# Autodesk Inventor assembly: Pendolo_Inverso
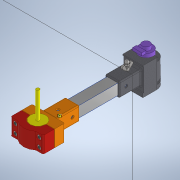
[picture p0: Inventor's stored thumbnail of the model, 180x180]
Saved by Autodesk Inventor 2020.2 (Build 242310000, 310)
## iProperties
Created: 2019-11-10
Part Number: Pendolo_Inverso
Document SubType Name: Assembly
Designer: socci
Mass: 329.019 g
Surface Area: 919.573 cm^2
Volume: 203.34 cm^3
Density: 1.61807 g/cm^3
Author: socci
## Documents named in this file (13)
- C:\Users\socci\Desktop\mv-Project\04_PartDraw\Assieme_Barra.iam
- C:\Users\socci\Desktop\mv-Project\04_PartDraw\Componenti\1_Asse_cuscinetti.ipt
- C:\Users\socci\Desktop\mv-Project\04_PartDraw\Componenti\2_Connettore_inf_sup.ipt
- C:\Users\socci\Desktop\mv-Project\04_PartDraw\Componenti\3_Connettore_inf_INF.ipt
- C:\Users\socci\Desktop\mv-Project\04_PartDraw\Componenti\4_barra.ipt
- C:\Users\socci\Desktop\mv-Project\04_PartDraw\Componenti\8_Connettore_sup.ipt
- C:\Users\socci\Desktop\mv-Project\04_PartDraw\Componenti\7_Motore.ipt
- C:\Users\socci\Documents\Inventor\Content Center Files\R2020\it-IT\ANSI B18.2.4.2M\ANSI B18.2.4.2M - M4x0,7 - 7.ipt
- C:\Users\socci\Documents\Inventor\Content Center Files\R2020\it-IT\ISO 7045  H\ISO 7045 - M4 x 40 - 4.8 - H - ISO.ipt
- C:\Users\socci\Documents\Inventor\Content Center Files\R2020\it-IT\ISO 7089\ISO 7089 - 4 - 140 HV(1).ipt
- C:\Users\socci\Documents\Inventor\Content Center Files\R2020\it-IT\ISO 4017(1)\ISO 4017 - M4 x 40 - ISO.ipt
- C:\Users\socci\Documents\Inventor\Content Center Files\R2020\it-IT\DIN 1587\DIN 1587 - M4 x 0,7.ipt
- C:\Users\socci\Documents\Inventor\Content Center Files\R2020\it-IT\JIS B 1185 T 1\JIS B 1185 - M4.ipt
## Components (26 placed, 12 different names)
1. 1_Asse_cuscinetti:1 — Inserimento:5, Inserimento:6
2. 2_Connettore_inf_sup:1 — Inserimento:6, Coincidente:1, Coincidente:5, Coincidente:6, Coincidente:7, Inserimento:12, Inserimento:13, Inserimento:14, Inserimento:15
3. 3_Connettore_inf_INF:1 — Inserimento:5, Coincidente:1, Inserimento:8, Coincidente:11, Inserimento:9, Coincidente:12, Inserimento:10, Coincidente:13, Inserimento:11, Coincidente:14, Inserimento:20, Inserimento:21, Inserimento:22, Inserimento:23, Tangente:1
4. 4_barra:1 — Coincidente:5, Coincidente:6, Coincidente:7, Coincidente:8, Coincidente:9, Coincidente:10, Coincidente:15, Coincidente:16
5. 8_Connettore_sup:1 — Coincidente:8, Coincidente:9, Coincidente:10, Inserimento:7, Inserimento:24, Inserimento:27
6. 7_Motore:1 — Inserimento:7
7. ANSI B18.2.4.2M M4x0,7:2 — Inserimento:11, Coincidente:14
8. ANSI B18.2.4.2M M4x0,7:3 — Inserimento:8, Coincidente:11
9. ANSI B18.2.4.2M M4x0,7:4 — Inserimento:10, Coincidente:13
10. ANSI B18.2.4.2M M4x0,7:5 — Inserimento:9, Coincidente:12
11. ISO 7045 H M4 x 40 - 4.8 - H:1 — Inserimento:13
12. ISO 7045 H M4 x 40 - 4.8 - H:2 — Inserimento:14
13. ISO 7045 H M4 x 40 - 4.8 - H:3 — Inserimento:12
14. ISO 7045 H M4 x 40 - 4.8 - H:4 — Inserimento:15
15. ISO 7089 4:1 — Inserimento:16, Inserimento:20
16. ISO 7089 4:2 — Inserimento:17, Inserimento:21
17. ISO 7089 4:3 — Inserimento:17
18. ISO 7089 4:4 — Inserimento:16
19. ISO 7089 4:5 — Inserimento:18, Inserimento:22
20. ISO 7089 4:6 — Inserimento:19
21. ISO 7089 4:7 — Inserimento:19, Inserimento:23
22. ISO 7089 4:8 — Inserimento:18
23. ISO 7089 4:9 — Inserimento:24, Inserimento:25
24. ISO 4017 M4 x 40:1 — Inserimento:25, Inserimento:26
25. DIN 1587 M4:1 — Inserimento:26
26. JIS B 1185 Tipo 1 - Metrico M4:1 — Inserimento:27
## Relationships (37: Insert 23, Mate 13, Tangent 1)
- Inserimento:5: 1_Asse_cuscinetti:1 ↔ 3_Connettore_inf_INF:1
- Inserimento:6: 1_Asse_cuscinetti:1 ↔ 2_Connettore_inf_sup:1
- Coincidente:1 [Mate] (1 mm): 2_Connettore_inf_sup:1 ↔ 3_Connettore_inf_INF:1
- Coincidente:5 [Mate] (0.5 mm): 2_Connettore_inf_sup:1 ↔ 4_barra:1
- Coincidente:6 [Mate] (0.5 mm): 2_Connettore_inf_sup:1 ↔ 4_barra:1
- Coincidente:7 [Mate]: 2_Connettore_inf_sup:1 ↔ 4_barra:1
- Coincidente:8 [Mate] (0.5 mm): 4_barra:1 ↔ 8_Connettore_sup:1
- Coincidente:9 [Mate] (0.5 mm): 4_barra:1 ↔ 8_Connettore_sup:1
- Coincidente:10 [Mate]: 4_barra:1 ↔ 8_Connettore_sup:1
- Inserimento:7: 8_Connettore_sup:1 ↔ 7_Motore:1
- Inserimento:8: 3_Connettore_inf_INF:1 ↔ ANSI B18.2.4.2M M4x0,7:3
- Coincidente:11 [Mate] (0.5 mm): 3_Connettore_inf_INF:1 ↔ ANSI B18.2.4.2M M4x0,7:3
- Inserimento:9: 3_Connettore_inf_INF:1 ↔ ANSI B18.2.4.2M M4x0,7:5
- Coincidente:12 [Mate] (0.5 mm): 3_Connettore_inf_INF:1 ↔ ANSI B18.2.4.2M M4x0,7:5
- Inserimento:10: 3_Connettore_inf_INF:1 ↔ ANSI B18.2.4.2M M4x0,7:4
- Coincidente:13 [Mate] (0.5 mm): 3_Connettore_inf_INF:1 ↔ ANSI B18.2.4.2M M4x0,7:4
- Inserimento:11: 3_Connettore_inf_INF:1 ↔ ANSI B18.2.4.2M M4x0,7:2
- Coincidente:14 [Mate] (0.5 mm): 3_Connettore_inf_INF:1 ↔ ANSI B18.2.4.2M M4x0,7:2
- Inserimento:12: 2_Connettore_inf_sup:1 ↔ ISO 7045 H M4 x 40 - 4.8 - H:3
- Inserimento:13: 2_Connettore_inf_sup:1 ↔ ISO 7045 H M4 x 40 - 4.8 - H:1
- Inserimento:14: 2_Connettore_inf_sup:1 ↔ ISO 7045 H M4 x 40 - 4.8 - H:2
- Inserimento:15: 2_Connettore_inf_sup:1 ↔ ISO 7045 H M4 x 40 - 4.8 - H:4
- Inserimento:16: ISO 7089 4:1 ↔ ISO 7089 4:4
- Inserimento:17: ISO 7089 4:2 ↔ ISO 7089 4:3
- Inserimento:18: ISO 7089 4:5 ↔ ISO 7089 4:8
- Inserimento:19: ISO 7089 4:6 ↔ ISO 7089 4:7
- Inserimento:20: 3_Connettore_inf_INF:1 ↔ ISO 7089 4:1
- Inserimento:21: 3_Connettore_inf_INF:1 ↔ ISO 7089 4:2
- Inserimento:22: 3_Connettore_inf_INF:1 ↔ ISO 7089 4:5
- Inserimento:23: 3_Connettore_inf_INF:1 ↔ ISO 7089 4:7
- Coincidente:15 [Mate] (-10 mm): 4_barra:1
- Coincidente:16 [Mate] (-10 mm): 4_barra:1
- Tangente:1: 3_Connettore_inf_INF:1
- Inserimento:24: 8_Connettore_sup:1 ↔ ISO 7089 4:9
- Inserimento:25: ISO 7089 4:9 ↔ ISO 4017 M4 x 40:1
- Inserimento:26: ISO 4017 M4 x 40:1 ↔ DIN 1587 M4:1
- Inserimento:27: 8_Connettore_sup:1 ↔ JIS B 1185 Tipo 1 - Metrico M4:1
